# Autodesk Inventor assembly: Assemlby_TIRFImager_v0
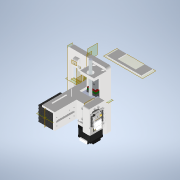
[picture p0: Inventor's stored thumbnail of the model, 180x180]
Saved by Autodesk Inventor 2022 (Build 260153000, 153)
## iProperties
Created: 2022-05-21
Part Number: Assemlby_TIRFImager_v0
Document SubType Name: Assembly
Designer: diederichbenedict
Author: diederichbenedict
## Documents named in this file (15)
- C:\Users\diederichbenedict\Dropbox\Dokumente\Promotion\PROJECTS\TIRFImager\INVENTOR\Assemlby_TIRFImager_50mmNEMA_v1.iam
- C:\Users\diederichbenedict\Dropbox\Dokumente\Promotion\PROJECTS\TIRFImager\INVENTOR\00_chipnano_waveguide_slidsize.ipt
- C:\Users\diederichbenedict\Dropbox\Dokumente\Promotion\PROJECTS\TIRFImager\INVENTOR\00_LASER_640nm.ipt
- C:\Users\diederichbenedict\Dropbox\Dokumente\Promotion\PROJECTS\TIRFImager\INVENTOR\00_KES400.iam
- C:\Users\diederichbenedict\Dropbox\Dokumente\Promotion\PROJECTS\TIRFImager\INVENTOR\30_XYTabel_Aliexpress_cellSTORM_chiptray_clamp.ipt
- C:\Users\diederichbenedict\Dropbox\Dokumente\Promotion\PROJECTS\TIRFImager\INVENTOR\TIRFImager_Laserbase_v1.ipt
- C:\Users\diederichbenedict\Dropbox\Dokumente\Promotion\PROJECTS\TIRFImager\INVENTOR\30_XYTabel_Aliexpress_cellSTORM_chiptray_spacer.ipt
- C:\Users\diederichbenedict\Dropbox\Dokumente\Promotion\PROJECTS\TIRFImager\INVENTOR\00_Linear_Stage_NEMA11_china.iam
- C:\Users\diederichbenedict\Dropbox\Dokumente\Promotion\PROJECTS\TIRFImager\INVENTOR\TIRFImager_base_50mm_NEMA11_v0.ipt
- C:\Users\diederichbenedict\Dropbox\Dokumente\Promotion\PROJECTS\TIRFImager\INVENTOR\00_Carriage.ipt
- C:\Users\diederichbenedict\Dropbox\Dokumente\Promotion\PROJECTS\TIRFImager\INVENTOR\00_Comar_Mirror.ipt
- C:\Users\diederichbenedict\Dropbox\Dokumente\Promotion\PROJECTS\TIRFImager\INVENTOR\ESP3-CAM v4.iam
- C:\Users\diederichbenedict\Dropbox\Dokumente\Promotion\PROJECTS\TIRFImager\INVENTOR\00_cctvlens.ipt
- C:\Users\diederichbenedict\Dropbox\Dokumente\Promotion\PROJECTS\TIRFImager\INVENTOR\30_ESP32_Camera_tray.ipt
- C:\Users\diederichbenedict\Dropbox\Dokumente\Promotion\PROJECTS\TIRFImager\INVENTOR\30_Cameraholder.ipt
## Components (15 placed, 14 different names)
1. TIRFImager_base_50mm_NEMA11_v0:1 — Passend:1, Fluchtend:1, Fluchtend:2, Fluchtend:3, Winkel:3, Einfügen:1, Einfügen:2, Passend:3, Fluchtend:4, Passend:4, Fluchtend:8, Fluchtend:9
2. 00_chipnano_waveguide_slidsize:1 — Passend:1, Fluchtend:1, Fluchtend:2
3. 00_KES400:1 [sub-assembly] — Fluchtend:3, Winkel:3, Fluchtend:5, Einfügen:3, Einfügen:4
4. 30_XYTabel_Aliexpress_cellSTORM_chiptray_clamp:1 — Einfügen:1
5. 30_XYTabel_Aliexpress_cellSTORM_chiptray_clamp:2 — Einfügen:2
6. 30_XYTabel_Aliexpress_cellSTORM_chiptray_spacer:1
7. 00_Linear_Stage_NEMA11_china:1 [sub-assembly] — Passend:3, Fluchtend:4, Passend:4, Passend:5, Passend:6
8. 00_LASER_640nm:1 — Fluchtend:5, Passend:5, Passend:7, Passend:8
9. TIRFImager_Laserbase_v1:1 — Einfügen:3, Einfügen:4, Passend:9, Einfügen:5, Fluchtend:6, Fluchtend:7
10. 00_Carriage:1 — Passend:6, Passend:7, Passend:8
11. 00_Comar_Mirror:1 — Passend:9
12. 00_cctvlens:1 — Einfügen:5, Passend:10
13. ESP3-CAM v4:1 [sub-assembly] — Passend:10, Winkel:4, Passend:11
14. 30_ESP32_Camera_tray:1 — Fluchtend:6, Fluchtend:7, Winkel:4, Passend:11
15. 30_Cameraholder:1 — Fluchtend:8, Fluchtend:9
## Relationships (27: Mate 11, Flush 9, Insert 5, Angle 2)
- Passend:1 [Mate]: TIRFImager_base_50mm_NEMA11_v0:1 ↔ 00_chipnano_waveguide_slidsize:1
- Fluchtend:1 [Flush] (1 mm): TIRFImager_base_50mm_NEMA11_v0:1 ↔ 00_chipnano_waveguide_slidsize:1
- Fluchtend:2 [Flush] (4 mm): TIRFImager_base_50mm_NEMA11_v0:1 ↔ 00_chipnano_waveguide_slidsize:1
- [Mate]: 00_chipnano_waveguide_slidsize:1 ↔ 00_KES400:1
- Fluchtend:3 [Flush] (3 mm): TIRFImager_base_50mm_NEMA11_v0:1 ↔ 00_KES400:1
- Winkel:3 [Angle] (0 deg): TIRFImager_base_50mm_NEMA11_v0:1 ↔ 00_KES400:1
- Einfügen:1 [Insert]: TIRFImager_base_50mm_NEMA11_v0:1 ↔ 30_XYTabel_Aliexpress_cellSTORM_chiptray_clamp:1
- Einfügen:2 [Insert]: TIRFImager_base_50mm_NEMA11_v0:1 ↔ 30_XYTabel_Aliexpress_cellSTORM_chiptray_clamp:2
- Passend:3 [Mate]: TIRFImager_base_50mm_NEMA11_v0:1 ↔ 00_Linear_Stage_NEMA11_china:1
- Fluchtend:4 [Flush]: TIRFImager_base_50mm_NEMA11_v0:1 ↔ 00_Linear_Stage_NEMA11_china:1
- Passend:4 [Mate]: TIRFImager_base_50mm_NEMA11_v0:1 ↔ 00_Linear_Stage_NEMA11_china:1
- Fluchtend:5 [Flush]: 00_KES400:1 ↔ 00_LASER_640nm:1
- Passend:5 [Mate] (20 mm): 00_Linear_Stage_NEMA11_china:1 ↔ 00_LASER_640nm:1
- Passend:6 [Mate]: 00_Linear_Stage_NEMA11_china:1 ↔ 00_Carriage:1
- Passend:7 [Mate]: 00_LASER_640nm:1 ↔ 00_Carriage:1
- Passend:8 [Mate] (7.5 mm): 00_LASER_640nm:1 ↔ 00_Carriage:1
- Einfügen:3 [Insert]: 00_KES400:1 ↔ TIRFImager_Laserbase_v1:1
- Einfügen:4 [Insert]: 00_KES400:1 ↔ TIRFImager_Laserbase_v1:1
- Passend:9 [Mate]: TIRFImager_Laserbase_v1:1 ↔ 00_Comar_Mirror:1
- Einfügen:5 [Insert] (-10 mm): TIRFImager_Laserbase_v1:1 ↔ 00_cctvlens:1
- Fluchtend:6 [Flush]: TIRFImager_Laserbase_v1:1 ↔ 30_ESP32_Camera_tray:1
- Fluchtend:7 [Flush]: TIRFImager_Laserbase_v1:1 ↔ 30_ESP32_Camera_tray:1
- Passend:10 [Mate]: 00_cctvlens:1 ↔ ESP3-CAM v4:1
- Winkel:4 [Angle] (0 deg): ESP3-CAM v4:1 ↔ 30_ESP32_Camera_tray:1
- Passend:11 [Mate] (12 mm): ESP3-CAM v4:1 ↔ 30_ESP32_Camera_tray:1
- Fluchtend:8 [Flush]: TIRFImager_base_50mm_NEMA11_v0:1 ↔ 30_Cameraholder:1
- Fluchtend:9 [Flush]: TIRFImager_base_50mm_NEMA11_v0:1 ↔ 30_Cameraholder:1
